# Autodesk Inventor assembly: Assembly
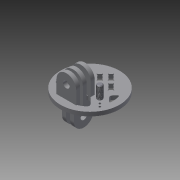
[picture p0: Inventor's stored thumbnail of the model, 180x180]
Saved by Autodesk Inventor 2014 SP1 (Build 180222100, 222)
## iProperties
Created: 2014-03-20
Part Number: Assembly
Document SubType Name: Assembly
Designer: ehagerup
Author: ehagerup
## Documents named in this file (5)
- C:\Users\ehagerup\SkyDrive\Documents\Mechanical Sketches\Animatronic Tail V4\Assembly.iam
- C:\Users\ehagerup\SkyDrive\Documents\Mechanical Sketches\Animatronic Tail V4\Segment.ipt
- C:\Users\ehagerup\SkyDrive\Documents\Mechanical Sketches\Animatronic Tail V4\Connector_3.ipt
- C:\Users\ehagerup\SkyDrive\Documents\Mechanical Sketches\Animatronic Tail V4\Connector_2.ipt
- C:\Users\ehagerup\Documents\Inventor\Content Center Files\R2014\en-US\JIS B 1180  A+B\JIS B 1180 - A + B M4x12x5.88 - 10.ipt
## Components (8 placed, 4 different names)
1. Segment:1 — Flush:7, Mate:1, Mate:3, Mate:4, Mate:5, Mate:6, Mate:9, Mate:10, Mate:11, Mate:12
2. Connector_3:1 — Flush:5, Flush:6, Mate:1, Mate:2, Mate:8
3. Connector_3:2 — Flush:5, Flush:6, Flush:7, Mate:7
4. Connector_2:1 — Flush:2, Flush:3, Mate:5, Mate:6, Mate:8
5. Connector_2:2 — Flush:1, Flush:2, Flush:3, Flush:4, Mate:4, Mate:7
6. Connector_2:3 — Flush:1, Flush:4, Mate:2, Mate:3
7. JIS B 1180 A+B - Metric A + B M4x12:1 — Mate:11, Mate:12
8. JIS B 1180 A+B - Metric A + B M4x12:2 — Mate:9, Mate:10
## Relationships (19: Mate 12, Flush 7)
- Flush:1: Connector_2:2 ↔ Connector_2:3
- Flush:2: Connector_2:1 ↔ Connector_2:2
- Flush:3: Connector_2:1 ↔ Connector_2:2
- Flush:4: Connector_2:2 ↔ Connector_2:3
- Flush:5: Connector_3:1 ↔ Connector_3:2
- Flush:6: Connector_3:1 ↔ Connector_3:2
- Flush:7: Segment:1 ↔ Connector_3:2
- Mate:1: Segment:1 ↔ Connector_3:1
- Mate:2: Connector_3:1 ↔ Connector_2:3
- Mate:3: Segment:1 ↔ Connector_2:3
- Mate:4: Segment:1 ↔ Connector_2:2
- Mate:5: Segment:1 ↔ Connector_2:1
- Mate:6: Segment:1 ↔ Connector_2:1
- Mate:7: Connector_3:2 ↔ Connector_2:2
- Mate:8: Connector_3:1 ↔ Connector_2:1
- Mate:9: Segment:1 ↔ JIS B 1180 A+B - Metric A + B M4x12:2
- Mate:10: Segment:1 ↔ JIS B 1180 A+B - Metric A + B M4x12:2
- Mate:11: Segment:1 ↔ JIS B 1180 A+B - Metric A + B M4x12:1
- Mate:12: Segment:1 ↔ JIS B 1180 A+B - Metric A + B M4x12:1
